# Autodesk Inventor assembly: RT_MAIN_A_001
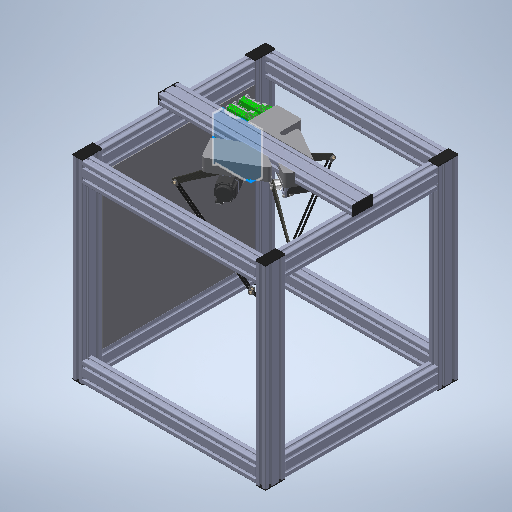
[picture p0: Inventor's stored thumbnail of the model, 512x512]
Saved by Autodesk Inventor 2025.4 (Build 294407000, 407)
## iProperties
Created: 2026-05-15
Part Number: RT_MAIN_A_001
Document SubType Name: Assembly
Designer: louis
Author: louis
## Documents named in this file (6)
- C:\Users\louis\OneDrive\Desktop\R_Trident\02_CAD\05_Top_Assembly\RT_MAIN_A_001.iam
- C:\Users\louis\OneDrive\Desktop\R_Trident\02_CAD\04_Subassemblies\RT_FRM_A_003_Frame.iam
- C:\Users\louis\OneDrive\Desktop\R_Trident\02_CAD\04_Subassemblies\RT_FRM_A_002_Dynamics.iam
- C:\Users\louis\OneDrive\Desktop\R_Trident\02_CAD\03_Parts_Custom\RT_FRM_MC_008_TopPlate_Support.ipt
- C:\Users\louis\OneDrive\Desktop\R_Trident\02_CAD\01_Standard_Parts\Electrical_Automation\WAGO_Din.iam
- C:\Users\louis\OneDrive\Desktop\R_Trident\02_CAD\01_Standard_Parts\A6-400EC\A6-400EC.iam
## Components (7 placed, 5 different names)
1. RT_FRM_A_003_Frame:1 [sub-assembly] — Flush:1, Flush:5, Mate:1, Mate:7, Mate:12, Mate:13, Mate:14, Mate:15, Mate:18, Mate:20, Mate:21, Mate:22, Mate:23, Mate:24, Mate:25, Mate:26
2. RT_FRM_A_002_Dynamics:1 [sub-assembly] — Flush:3, Flush:4, Flush:5, Mate:9, Mate:10, Mate:11
3. RT_FRM_MC_008_TopPlate_Support:1 — Mate:9, Mate:10, Mate:11
4. WAGO_Din:1 [sub-assembly] — Mate:12, Mate:13, Mate:18, Mate:19, Mate:20
5. A6-400EC:1 [sub-assembly] — Mate:21, Mate:22
6. A6-400EC:2 [sub-assembly] — Mate:23, Mate:24
7. A6-400EC:3 [sub-assembly] — Mate:25, Mate:26
## Relationships (24: Mate 20, Flush 4)
- Flush:1: RT_FRM_A_003_Frame:1
- Flush:3: RT_FRM_A_002_Dynamics:1
- Flush:4: RT_FRM_A_002_Dynamics:1
- Flush:5: RT_FRM_A_003_Frame:1 ↔ RT_FRM_A_002_Dynamics:1
- Mate:1: RT_FRM_A_003_Frame:1
- Mate:7: RT_FRM_A_003_Frame:1
- Mate:9: RT_FRM_A_002_Dynamics:1 ↔ RT_FRM_MC_008_TopPlate_Support:1
- Mate:10: RT_FRM_A_002_Dynamics:1 ↔ RT_FRM_MC_008_TopPlate_Support:1
- Mate:11: RT_FRM_A_002_Dynamics:1 ↔ RT_FRM_MC_008_TopPlate_Support:1
- Mate:12: RT_FRM_A_003_Frame:1 ↔ WAGO_Din:1
- Mate:13: RT_FRM_A_003_Frame:1 ↔ WAGO_Din:1
- Mate:14: RT_FRM_A_003_Frame:1
- Mate:15: RT_FRM_A_003_Frame:1
- Mate:16
- Mate:17
- Mate:18: RT_FRM_A_003_Frame:1 ↔ WAGO_Din:1
- Mate:19: WAGO_Din:1
- Mate:20: RT_FRM_A_003_Frame:1 ↔ WAGO_Din:1
- Mate:21: RT_FRM_A_003_Frame:1 ↔ A6-400EC:1
- Mate:22: RT_FRM_A_003_Frame:1 ↔ A6-400EC:1
- Mate:23: RT_FRM_A_003_Frame:1 ↔ A6-400EC:2
- Mate:24: RT_FRM_A_003_Frame:1 ↔ A6-400EC:2
- Mate:25: RT_FRM_A_003_Frame:1 ↔ A6-400EC:3
- Mate:26: RT_FRM_A_003_Frame:1 ↔ A6-400EC:3
